# Autodesk Inventor assembly: Beam_stempel_beslag
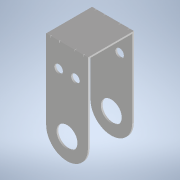
[picture p0: Inventor's stored thumbnail of the model, 180x180]
Saved by Autodesk Inventor 2022 (Build 260153000, 153)
## iProperties
Created: 2022-04-28
Part Number: Beam_stempel_beslag
Document SubType Name: Assembly
Designer: patri
Author: patri
## Documents named in this file (3)
- H:\OneDrive - Syddansk Universitet\2. Semester Master\Mekaniske Elementer\Mini Project\2020-10-23\Workspaces\Workspace\Beslag_beam_cylinder\Beam_stempel_beslag.iam
- H:\OneDrive - Syddansk Universitet\2. Semester Master\Mekaniske Elementer\Mini Project\2020-10-23\Workspaces\Workspace\Beslag_beam_cylinder\backstop_beslag.ipt
- H:\OneDrive - Syddansk Universitet\2. Semester Master\Mekaniske Elementer\Mini Project\2020-10-23\Workspaces\Workspace\Beslag_beam_cylinder\side_beslag.ipt
## Components (3 placed, 2 different names)
1. backstop_beslag:1 — Rigid:1, Rigid:2
2. side_beslag:1 — Rigid:1
3. side_beslag:2 — Rigid:2
## Relationships (2: WeldJoint 2)
- Rigid:1 [WeldJoint]: backstop_beslag:1 ↔ side_beslag:1
- Rigid:2 [WeldJoint]: backstop_beslag:1 ↔ side_beslag:2
